# Autodesk Inventor assembly: Peristaltic pump with extension
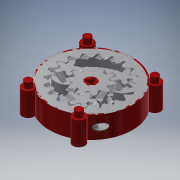
[picture p0: Inventor's stored thumbnail of the model, 180x180]
Saved by Autodesk Inventor 2017 (Build 210142000, 142)
## iProperties
Created: 2016-11-08
Part Number: Peristaltic pump with extension
Document SubType Name: Assembly
Designer: Camilo
Author: Camilo
## Documents named in this file (3)
- Z:\Github\AgingTests\3D parts\Peristaltic pump adapter\Peristaltic pump with extension.iam
- Z:\Github\AgingTests\3D parts\Peristaltic pump adapter\Peristaltic Pump.ipt
- Z:\Github\AgingTests\3D parts\Peristaltic pump adapter\peristalticPumpExtension_scaled.ipt
## Components (2 placed, 2 different names)
1. Peristaltic Pump:1 — Mate:1, Angle:1
2. peristalticPumpExtension_scaled:1 — Mate:1, Angle:1
## Relationships (2: Mate 1, Angle 1)
- Mate:1: Peristaltic Pump:1 ↔ peristalticPumpExtension_scaled:1
- Angle:1 (180 deg): Peristaltic Pump:1 ↔ peristalticPumpExtension_scaled:1
